# Autodesk Inventor assembly: Rb oven housing
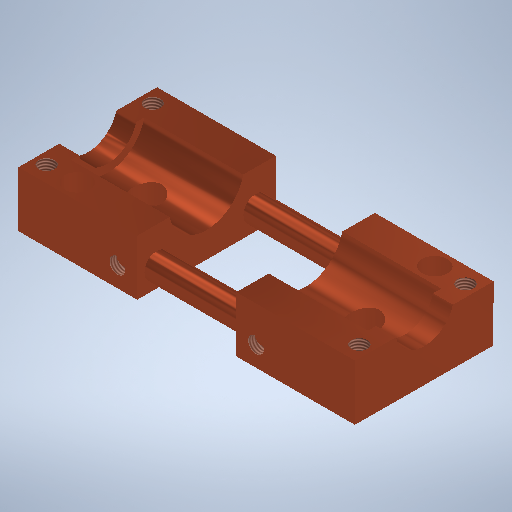
[picture p0: Inventor's stored thumbnail of the model, 512x512]
Saved by Autodesk Inventor 2025.3 (Build 293356000, 356)
## iProperties
Created: 2025-04-24
Part Number: Rb oven housing
Document SubType Name: Assembly
Designer: E. Moreno
Author: E. Moreno
Title: Carcasa Horno - Ensamblado
## Documents named in this file (4)
- E:\Users\USER\Documents\GitHub\LAFriOC\Rb oven\Rb oven housing\Modificación\Rb oven housing - Bottom.iam
- E:\Users\USER\Documents\GitHub\LAFriOC\Rb oven\Rb oven housing\Modificación\Rb oven housing bottom-back_front.ipt
- E:\Users\USER\Documents\GitHub\LAFriOC\Rb oven\Rb oven housing\Modificación\Rb oven housing post.ipt
- E:\Users\USER\Documents\GitHub\LAFriOC\Rb oven\Rb oven housing\Modificación\Rb oven housing bottom-back_front_MIR_MIR.ipt
## Components (4 placed, 3 different names)
1. Rb oven housing bottom-back_front:1 — Mate:1, Insert:1
2. Rb oven housing post:1 — Insert:1
3. Rb oven housing post:2 — Mate:1, Insert:2
4. Rb oven housing bottom-back_front_MIR_MIR:1 — Insert:2
## Relationships (3: Insert 2, Mate 1)
- Mate:1: Rb oven housing bottom-back_front:1 ↔ Rb oven housing post:2
- Insert:1 (-15 mm): Rb oven housing bottom-back_front:1 ↔ Rb oven housing post:1
- Insert:2 (-15 mm): Rb oven housing post:2 ↔ Rb oven housing bottom-back_front_MIR_MIR:1
